# Autodesk Inventor assembly: Assembly1
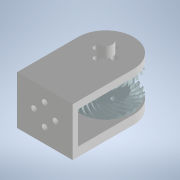
[picture p0: Inventor's stored thumbnail of the model, 180x180]
Saved by Autodesk Inventor 2022 (Build 260153000, 153)
## iProperties
Created: 2022-04-18
Part Number: Assembly1
Document SubType Name: Assembly
Designer: Mlees
Author: Mlees
## Documents named in this file (4)
- C:\Users\Mlees\Desktop\504Engineering\Project_0000\Designs\Design_1\Created_Parts\Assembly1.iam
- C:\Users\Mlees\Desktop\504Engineering\Project_0000\Designs\Design_1\Created_Parts\Spiral Bevel gear Z2.ipt
- C:\Users\Mlees\Desktop\504Engineering\Project_0000\Designs\Design_1\Created_Parts\Spiral Bevel gear Z2_Right.ipt
- C:\Users\Mlees\Desktop\504Engineering\Project_0000\Designs\Design_1\Created_Parts\Base_Mount.ipt
## Components (3 placed, 3 different names)
1. Spiral Bevel gear Z2:1 — Mate:3, Mate:4
2. Spiral Bevel gear Z2_Right:1 — Mate:1, Mate:2
3. Base_Mount:1 — Mate:1, Mate:2, Mate:3, Mate:4
## Relationships (4: Mate 4)
- Mate:1: Spiral Bevel gear Z2_Right:1 ↔ Base_Mount:1
- Mate:2: Spiral Bevel gear Z2_Right:1 ↔ Base_Mount:1
- Mate:3: Spiral Bevel gear Z2:1 ↔ Base_Mount:1
- Mate:4: Spiral Bevel gear Z2:1 ↔ Base_Mount:1
